# Autodesk Inventor assembly: AM14U3 Square Frame Half
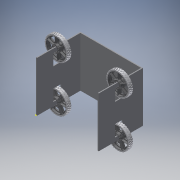
[picture p0: Inventor's stored thumbnail of the model, 180x180]
Saved by Autodesk Inventor 2018 (Build 220112000, 112)
## iProperties
Created: 2018-01-13
Part Number: AM14U3 Square Frame Half
Document SubType Name: Assembly
Designer: 21alebarron
Author: 21alebarron
## Documents named in this file (3)
- C:\Users\21alebarron\Documents\GitHub\RobotDesigns2018\AM14U3 Square Frame Half.iam
- H:\DDP\trammel\Part73.ipt
- H:\DDP\6 HiGrip Asm Rev II.0001.iam
## Components (5 placed, 2 different names)
1. Part73:1 — Mate:1, Mate:2, Mate:3, Mate:4, Mate:5, Mate:6, Mate:7, Mate:8
2. 6 HiGrip Asm Rev II.0001:1 [sub-assembly] — Mate:3, Mate:8
3. 6 HiGrip Asm Rev II.0001:2 [sub-assembly] — Mate:4, Mate:5
4. 6 HiGrip Asm Rev II.0001:3 [sub-assembly] — Mate:2, Mate:6
5. 6 HiGrip Asm Rev II.0001:4 [sub-assembly] — Mate:1, Mate:7
## Relationships (8: Mate 8)
- Mate:1: Part73:1 ↔ 6 HiGrip Asm Rev II.0001:4
- Mate:2: Part73:1 ↔ 6 HiGrip Asm Rev II.0001:3
- Mate:3: Part73:1 ↔ 6 HiGrip Asm Rev II.0001:1
- Mate:4: Part73:1 ↔ 6 HiGrip Asm Rev II.0001:2
- Mate:5: Part73:1 ↔ 6 HiGrip Asm Rev II.0001:2
- Mate:6: Part73:1 ↔ 6 HiGrip Asm Rev II.0001:3
- Mate:7: Part73:1 ↔ 6 HiGrip Asm Rev II.0001:4
- Mate:8: Part73:1 ↔ 6 HiGrip Asm Rev II.0001:1
